# Autodesk Inventor assembly: Pully25mmx12mm
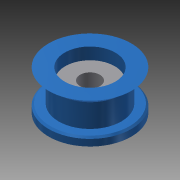
[picture p0: Inventor's stored thumbnail of the model, 180x180]
Saved by Autodesk Inventor 2013 (Build 170138000, 138)
## iProperties
Created: 2017-01-25
Part Number: Pully25mmx12mm
Document SubType Name: Assembly
Designer: Herman de Vries
Author: Herman de Vries
## Documents named in this file (3)
- D:\Projects\Inventor\PaintBoid_2\Pully25mmx12mm.iam
- D:\Projects\Inventor\PaintBoid_2\bearing 6mmx15mmx5mm.ipt
- D:\Projects\Inventor\PaintBoid_2\pully 15mmx25mmx12mm.ipt
## Components (2 placed, 2 different names)
1. bearing 6mmx15mmx5mm:1 — Insert:1
2. pully 15mmx25mmx12mm:1 — Insert:1
## Relationships (1: Insert 1)
- Insert:1 (-3.5 mm): bearing 6mmx15mmx5mm:1 ↔ pully 15mmx25mmx12mm:1
